# Autodesk Inventor assembly: still pipe
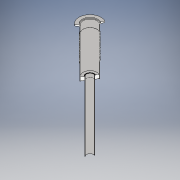
[picture p0: Inventor's stored thumbnail of the model, 180x180]
Saved by Autodesk Inventor 2018 (Build 220112000, 112)
## iProperties
Created: 2019-01-14
Part Number: still pipe
Document SubType Name: Assembly
Designer: Admin
Author: Admin
## Documents named in this file (10)
- C:\Users\Admin\Documents\Cryostat\CAD\still pipe.iam
- C:\Users\Admin\Documents\Cryostat\CAD\KF50 bellows.ipt
- C:\Users\Admin\Documents\Cryostat\CAD\universal connector.ipt
- C:\Users\Admin\Documents\Cryostat\CAD\1in ss pipe.ipt
- C:\Users\Admin\Documents\Cryostat\CAD\0in5 ss pipe.ipt
- C:\Users\Admin\Documents\Cryostat\CAD\brassbushing.ipt
- C:\Users\Admin\Documents\Cryostat\CAD\adapter.ipt
- C:\Users\Admin\Documents\Cryostat\CAD\heatsink.ipt
- C:\Users\Admin\Documents\Cryostat\CAD\pipeshift.ipt
- C:\Users\Admin\Documents\Cryostat\CAD\plug.ipt
## Components (9 placed, 9 different names)
1. KF50 bellows:1 — Mate:16, Flush:2
2. universal connector:1 — Mate:12, Mate:13
3. 1in ss pipe:3 — Mate:15, Flush:1, Mate:17, Mate:20, Mate:22
4. 0in5 ss pipe:1 — Mate:11, Mate:13, Mate:14, Mate:21, Mate:23
5. brassbushing:1 — Mate:11, Mate:12, Mate:14
6. adapter:1 — Mate:15, Flush:1, Mate:16, Flush:2, Mate:18, Mate:19
7. heatsink:1 — Mate:17, Mate:18, Mate:19
8. pipeshift:1 — Mate:20, Mate:21, Mate:22, Mate:23, Mate:24, Mate:25
9. plug:1 — Mate:24, Mate:25
## Relationships (17: Mate 15, Flush 2)
- Mate:11: 0in5 ss pipe:1 ↔ brassbushing:1
- Mate:12: universal connector:1 ↔ brassbushing:1
- Mate:13 (5.08 mm): universal connector:1 ↔ 0in5 ss pipe:1
- Mate:14 (-10.16 mm): 0in5 ss pipe:1 ↔ brassbushing:1
- Mate:15: 1in ss pipe:3 ↔ adapter:1
- Flush:1: 1in ss pipe:3 ↔ adapter:1
- Mate:16: KF50 bellows:1 ↔ adapter:1
- Flush:2: KF50 bellows:1 ↔ adapter:1
- Mate:17: 1in ss pipe:3 ↔ heatsink:1
- Mate:18: adapter:1 ↔ heatsink:1
- Mate:19: adapter:1 ↔ heatsink:1
- Mate:20: 1in ss pipe:3 ↔ pipeshift:1
- Mate:21: 0in5 ss pipe:1 ↔ pipeshift:1
- Mate:22: 1in ss pipe:3 ↔ pipeshift:1
- Mate:23: 0in5 ss pipe:1 ↔ pipeshift:1
- Mate:24: pipeshift:1 ↔ plug:1
- Mate:25: pipeshift:1 ↔ plug:1
